# Autodesk Inventor assembly: Fingertech Mini Power Switch
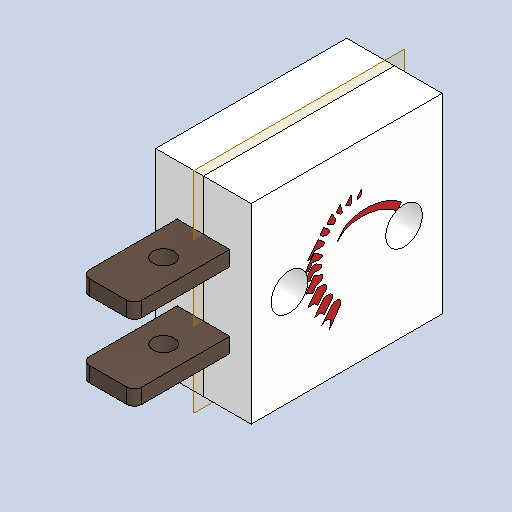
[picture p0: Inventor's stored thumbnail of the model, 512x512]
Saved by Autodesk Inventor 2023 (Build 270158000, 158)
## iProperties
Created: 2013-12-27
Part Number: Fingertech Mini Power Switch
Description: STEP AP214
Document SubType Name: Assembly
Designer: Nathan Cai
Mass: 2.15 g
Surface Area: 16.778 cm^2
Volume: 0.993186 cm^3
Density: 2.16475 g/cm^3
Sending System: SolidWorks 2014
Preprocessor: SwSTEP 2.0
Title: Fingertech Mini Power Switch.STEP
Revision Number: ANY
## Documents named in this file (4)
- D:\Inventor\Moon Cake V0.6\Fingertech Power Switch\Fingertech Mini Power Switch.iam
- D:\Inventor\Moon Cake V0.6\Fingertech Power Switch\PART A.ipt
- D:\Inventor\Moon Cake V0.6\Fingertech Power Switch\socket head cap screw_ai_HX-SHCS 0.086-56x0.375x0.375-S.ipt
- D:\Inventor\Moon Cake V0.6\Fingertech Power Switch\TERMINAL.ipt
## Components (5 placed, 5 different names)
1. PART A_1 — Symmetry:1
2. PART A_2 — Symmetry:1
3. socket head cap screw_ai_HX-SHCS 0.086-56x0.375x0.375-S_3
4. TERMINAL_4
5. TERMINAL_5
## Relationships (1: Symmetry 1)
- Symmetry:1: PART A_1 ↔ PART A_2
